# Autodesk Inventor assembly: Selection_Assy 2 Lanes
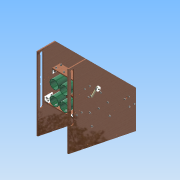
[picture p0: Inventor's stored thumbnail of the model, 180x180]
Saved by Autodesk Inventor 2018.1 (Build 221171000, 171)
## iProperties
Created: 2019-02-07
Part Number: Selection_Assy 2 Lanes
Document SubType Name: Assembly
Designer: James
Author: James
## Documents named in this file (24)
- C:\Users\admin\Desktop\Ball-Machine\Selection Sort\Selection - 2 Lanes\Selection_Assy 2 Lanes.iam
- C:\Users\admin\Desktop\Ball-Machine\Selection Sort\Selection_LHS.ipt
- C:\Users\admin\Desktop\Ball-Machine\Timing Gate\SAFL212 Oval 2 Bolt Flanged Unit.ipt
- C:\Users\admin\Desktop\Ball-Machine\Timing Gate\Nyloc Nut - M4.ipt
- C:\Users\admin\Desktop\Ball-Machine\Timing Gate\Socket Cap Screw - Standard - (A2) - M4 x 16.ipt
- C:\Users\admin\Desktop\Ball-Machine\Selection Sort\Locknut - M3.ipt
- C:\Users\admin\Desktop\Ball-Machine\Selection Sort\Socket Cap Screw - Standard - (A2) - M3 x 16.ipt
- C:\Users\admin\Desktop\Ball-Machine\Selection Sort\Selection_Lever 1.ipt
- C:\Users\admin\Desktop\Ball-Machine\Selection Sort\Socket Cap Screw - Standard - (A2) - M4 x 20.ipt
- C:\Users\admin\Desktop\Ball-Machine\Selection Sort\Selection_Lever Mount Piece.ipt
- C:\Users\admin\Desktop\Ball-Machine\Selection Sort\Socket Cap Screw - Standard - (A2) - M3 x 8.ipt
- C:\Users\admin\Desktop\Ball-Machine\Selection Sort\Selection_Washer.ipt
- C:\Users\admin\Desktop\Ball-Machine\Selection Sort\Selection_Gear 1.ipt
- C:\Users\admin\Desktop\Ball-Machine\Selection Sort\Selection_Lever 3.ipt
- C:\Users\admin\Desktop\Ball-Machine\Selection Sort\Selection_Counterweight.ipt
- C:\Users\admin\Desktop\Ball-Machine\Selection Sort\M3 x 20 - Hex. Head Set Screw (MS).ipt
- C:\Users\admin\Desktop\Ball-Machine\Selection Sort\Selection_Weight.ipt
- C:\Users\admin\Desktop\Ball-Machine\Selection Sort\Selection_Lever 2.ipt
- C:\Users\admin\Desktop\Ball-Machine\Selection Sort\Selection_Wire.ipt
- C:\Users\admin\Desktop\Ball-Machine\Selection Sort\Selection - 2 Lanes\Selection_Ramp 1 2 Lanes.iam
- C:\Users\admin\Desktop\Ball-Machine\Selection Sort\Selection - 2 Lanes\Selection_Exit Pipe Assy 2 Lanes.iam
- C:\Users\admin\Desktop\Ball-Machine\Selection Sort\Selection - 2 Lanes\Selection_Shaft Assy 2 Lanes.iam
- C:\Users\admin\Desktop\Ball-Machine\Timing Gate\Timing - 2 Lanes\Timing_Assy 2 Lanes.iam
- C:\Users\admin\Desktop\Ball-Machine\Selection Sort\Selection - 2 Lanes\Selection_Exit Pipe Assy Long 2 Lanes.iam
## Components (101 placed, 23 different names)
1. Selection_LHS:1 — Flush:1, Flush:2, Flush:3, Mate:4, Flush:9, Flush:10, Mate:37, Mate:38, Mate:39, Mate:42, Mate:43, Mate:56, Mate:70, Mate:71, Mate:116, Mate:117, Mate:118, Mate:119, Mate:120, Mate:121, Mate:128, Mate:129, Mate:131, Mate:152, Mate:155, Mate:193, Mate:194, Mate:195, Mate:196, Mate:200, Mate:203, Mate:204, Mate:205, Mate:206, Mate:207, Mate:208, Mate:210, Mate:211, Mate:213, Mate:214, Mate:225, Mate:226, Mate:227, Mate:228, Mate:232, Mate:233, Mate:234
2. Selection_Ramp 1 2 Lanes:1 [sub-assembly] — Flush:7, Mate:9, Mate:74, Mate:75, Mate:80, Mate:81, Mate:86, Mate:87, Mate:96, Mate:97, Mate:98, Mate:99
3. Selection_Ramp 1 2 Lanes:2 [sub-assembly] — Mate:4, Mate:76, Mate:77, Mate:82, Mate:83, Mate:88, Mate:89, Mate:94, Mate:95, Mate:102, Mate:103
4. Selection_Ramp 1 2 Lanes:3 [sub-assembly] — Flush:8, Mate:78, Mate:79, Mate:84, Mate:85, Mate:90, Mate:91, Mate:92, Mate:93, Mate:100, Mate:101
5. Selection_LHS:2 — Mate:9, Flush:9, Flush:10, Mate:52, Mate:53, Mate:54, Mate:55, Mate:57, Mate:62, Mate:63, Mate:74, Mate:75, Mate:76, Mate:77, Mate:78, Mate:79, Mate:104, Mate:105, Mate:106, Mate:107, Mate:108, Mate:109, Mate:132, Mate:134, Mate:135, Mate:148, Mate:149, Mate:159, Mate:160, Mate:161, Mate:162, Mate:163, Mate:164, Mate:189, Mate:190, Mate:191, Mate:192, Mate:197
6. Timing_Assy 2 Lanes:1 [sub-assembly] — Mate:36, Mate:37, Mate:38, Mate:39, Mate:40, Mate:41, Mate:44, Mate:45, Mate:48, Mate:49, Mate:50, Mate:51, Mate:56, Mate:57, Mate:58, Mate:59, Mate:60, Mate:61, Mate:66, Mate:67, Mate:68, Mate:69, Mate:219, Mate:220
7. SAFL212 Oval 2 Bolt Flanged Unit:3 — Mate:128, Mate:129, Mate:131, Mate:150, Mate:151, Mate:153, Mate:154, Mate:198
8. SAFL212 Oval 2 Bolt Flanged Unit:4 — Mate:132, Mate:134, Mate:135, Mate:144, Mate:145, Mate:146, Mate:147
9. Selection_Exit Pipe Assy Long 2 Lanes:1 [sub-assembly] — Mate:162, Mate:163, Mate:164, Mate:175, Mate:176, Mate:177, Mate:178, Mate:181, Mate:182, Mate:183, Mate:184
10. Selection_Exit Pipe Assy 2 Lanes:2 [sub-assembly] — Mate:159, Mate:160, Mate:161, Mate:173, Mate:174, Mate:179, Mate:180, Mate:185, Mate:186, Mate:187, Mate:188
11. Selection_Shaft Assy 2 Lanes:1 [sub-assembly] — Mate:197, Flush:11, Mate:198, Mate:247, Mate:248, Angle:1, Angle:2, Mate:249, Mate:250, Angle:3
12. Selection_Lever 1:1 — Mate:200, Mate:209, Mate:212, Flush:12, Mate:252, Flush:13
13. Selection_Lever Mount Piece:1 — Mate:209, Mate:210, Mate:211, Mate:212, Mate:215, Mate:216, Mate:217
14. Selection_Washer:1 — Mate:216, Mate:217, Mate:218
15. Selection_Gear 1:1 — Mate:219, Mate:220
16. Selection_Lever Mount Piece:2 — Mate:226, Mate:228, Mate:229, Mate:230
17. Socket Cap Screw - Standard - (A2) - M3 x 8:3 — Mate:225, Mate:227
18. Socket Cap Screw - Standard - (A2) - M3 x 8:4
19. Selection_Washer:2
20. Selection_Lever 3:1 — Mate:229, Mate:230, Tangent:3, Mate:251
21. Locknut - M3:9 — Mate:234
22. Socket Cap Screw - Standard - (A2) - M3 x 16:9 — Mate:232, Mate:233, Tangent:3
23. Selection_Counterweight:1 — Mate:235, Mate:236, Mate:242, Mate:247, Mate:248, Angle:1, Angle:2
24. Hex. Head Set Screw (MS) - M3 x 10:1 — Mate:235, Mate:236, Mate:237, Mate:238, Mate:239, Mate:240, Mate:241
25. Selection_Weight:1 — Mate:241, Mate:242, Mate:243
26. Selection_Weight:2 — Mate:240, Mate:243, Mate:244
27. Selection_Weight:3 — Mate:239, Mate:245, Mate:246
28. Selection_Weight:4 — Mate:238, Mate:244, Mate:245
29. Locknut - M3:10 — Mate:237, Mate:246
30. Selection_Lever 2:1 — Mate:249, Mate:250, Flush:12, Angle:3, Tangent:6, Tangent:7
31. Selection_Wire:1 — Mate:251, Mate:252, Flush:13
32. Socket Cap Screw - Standard - (A2) - M3 x 8:2 — Mate:215, Mate:218
33. Socket Cap Screw - Standard - (A2) - M3 x 8:1 — Mate:213, Mate:214
34. Nyloc Nut - M4:25 — Mate:207
35. Socket Cap Screw - Standard - (A2) - M4 x 20:2 — Mate:203, Mate:204, Tangent:6
36. Nyloc Nut - M4:26 — Mate:208
37. Socket Cap Screw - Standard - (A2) - M4 x 20:1 — Mate:205, Mate:206, Tangent:7
38. Nyloc Nut - M4:17 — Mate:173, Mate:179
39. Socket Cap Screw - Standard - (A2) - M4 x 16:17 — Mate:195
40. Nyloc Nut - M4:18 — Mate:174, Mate:180
41. Socket Cap Screw - Standard - (A2) - M4 x 16:18 — Mate:196
42. Nyloc Nut - M4:19 — Mate:175, Mate:176
43. Socket Cap Screw - Standard - (A2) - M4 x 16:19 — Mate:193
44. Nyloc Nut - M4:20 — Mate:177, Mate:178
45. Socket Cap Screw - Standard - (A2) - M4 x 16:20 — Mate:194
46. Nyloc Nut - M4:21 — Mate:181, Mate:183
47. Socket Cap Screw - Standard - (A2) - M4 x 16:21 — Mate:189
48. Nyloc Nut - M4:22 — Mate:182, Mate:184
49. Socket Cap Screw - Standard - (A2) - M4 x 16:22 — Mate:190
50. Nyloc Nut - M4:23 — Mate:185, Mate:188
51. Socket Cap Screw - Standard - (A2) - M4 x 16:23 — Mate:192
52. Nyloc Nut - M4:24 — Mate:186, Mate:187
53. Socket Cap Screw - Standard - (A2) - M4 x 16:24 — Mate:191
54. Locknut - M3:5 — Mate:149
55. Socket Cap Screw - Standard - (A2) - M3 x 16:5 — Mate:144, Mate:145
56. Locknut - M3:6 — Mate:148
57. Socket Cap Screw - Standard - (A2) - M3 x 16:6 — Mate:146, Mate:147
58. Locknut - M3:7 — Mate:152
59. Socket Cap Screw - Standard - (A2) - M3 x 16:7 — Mate:150, Mate:151
60. Locknut - M3:8 — Mate:155
61. Socket Cap Screw - Standard - (A2) - M3 x 16:8 — Mate:153, Mate:154
62. Nyloc Nut - M4:1 — Mate:44, Mate:46
63. Socket Cap Screw - Standard - (A2) - M4 x 16:1 — Mate:41, Mate:43, Mate:47
64. Nyloc Nut - M4:2 — Mate:45, Mate:47
65. Socket Cap Screw - Standard - (A2) - M4 x 16:2 — Mate:40, Mate:42, Mate:46
66. Nyloc Nut - M4:3 — Mate:49, Mate:50
67. Socket Cap Screw - Standard - (A2) - M4 x 16:3 — Mate:53, Mate:54
68. Nyloc Nut - M4:4 — Mate:48, Mate:51
69. Socket Cap Screw - Standard - (A2) - M4 x 16:4 — Mate:52, Mate:55
70. Locknut - M3:1 — Mate:62, Mate:64
71. Socket Cap Screw - Standard - (A2) - M3 x 16:1 — Mate:58, Mate:60, Mate:64
72. Locknut - M3:2 — Mate:63, Mate:65
73. Socket Cap Screw - Standard - (A2) - M3 x 16:2 — Mate:59, Mate:61, Mate:65
74. Locknut - M3:3 — Mate:70, Mate:72
75. Socket Cap Screw - Standard - (A2) - M3 x 16:3 — Mate:66, Mate:67, Mate:72
76. Locknut - M3:4 — Mate:71, Mate:73
77. Socket Cap Screw - Standard - (A2) - M3 x 16:4 — Mate:68, Mate:69, Mate:73
78. Nyloc Nut - M4:5 — Mate:104, Mate:110
79. Socket Cap Screw - Standard - (A2) - M4 x 16:5 — Mate:80, Mate:98, Mate:110
80. Nyloc Nut - M4:6 — Mate:105, Mate:112
81. Socket Cap Screw - Standard - (A2) - M4 x 16:6 — Mate:82, Mate:103, Mate:112
82. Nyloc Nut - M4:7 — Mate:106, Mate:115
83. Socket Cap Screw - Standard - (A2) - M4 x 16:7 — Mate:83, Mate:102, Mate:113
84. Nyloc Nut - M4:8 — Mate:107, Mate:113
85. Socket Cap Screw - Standard - (A2) - M4 x 16:8 — Mate:84, Mate:101, Mate:115
86. Nyloc Nut - M4:9 — Mate:108, Mate:111
87. Socket Cap Screw - Standard - (A2) - M4 x 16:9 — Mate:90, Mate:92, Mate:125
88. Nyloc Nut - M4:10 — Mate:109, Mate:114
89. Socket Cap Screw - Standard - (A2) - M4 x 16:10 — Mate:85, Mate:100, Mate:114
90. Nyloc Nut - M4:11 — Mate:116, Mate:124
91. Socket Cap Screw - Standard - (A2) - M4 x 16:11 — Mate:81, Mate:99, Mate:111
92. Nyloc Nut - M4:12 — Mate:117, Mate:126
93. Socket Cap Screw - Standard - (A2) - M4 x 16:12 — Mate:86, Mate:96, Mate:122
94. Nyloc Nut - M4:13 — Mate:118, Mate:127
95. Socket Cap Screw - Standard - (A2) - M4 x 16:13 — Mate:87, Mate:97, Mate:124
96. Nyloc Nut - M4:14 — Mate:119, Mate:125
97. Socket Cap Screw - Standard - (A2) - M4 x 16:14 — Mate:88, Mate:95, Mate:123
98. Nyloc Nut - M4:15 — Mate:120, Mate:123
99. Socket Cap Screw - Standard - (A2) - M4 x 16:15 — Mate:89, Mate:94, Mate:127
100. Nyloc Nut - M4:16 — Mate:121, Mate:122
101. Socket Cap Screw - Standard - (A2) - M4 x 16:16 — Mate:91, Mate:93, Mate:126
## Relationships (225: Mate 209, Flush 10, Tangent 3, Angle 3)
- Flush:1: Selection_LHS:1
- Flush:2: Selection_LHS:1
- Flush:3: Selection_LHS:1
- Flush:7: Selection_Ramp 1 2 Lanes:1
- Mate:4: Selection_LHS:1 ↔ Selection_Ramp 1 2 Lanes:2
- Flush:8: Selection_Ramp 1 2 Lanes:3
- Mate:9: Selection_Ramp 1 2 Lanes:1 ↔ Selection_LHS:2
- Flush:9: Selection_LHS:1 ↔ Selection_LHS:2
- Flush:10: Selection_LHS:1 ↔ Selection_LHS:2
- Mate:36: Timing_Assy 2 Lanes:1
- Mate:37: Selection_LHS:1 ↔ Timing_Assy 2 Lanes:1
- Mate:38: Selection_LHS:1 ↔ Timing_Assy 2 Lanes:1
- Mate:39: Selection_LHS:1 ↔ Timing_Assy 2 Lanes:1
- Mate:40: Timing_Assy 2 Lanes:1 ↔ Socket Cap Screw - Standard - (A2) - M4 x 16:2
- Mate:41: Timing_Assy 2 Lanes:1 ↔ Socket Cap Screw - Standard - (A2) - M4 x 16:1
- Mate:42: Selection_LHS:1 ↔ Socket Cap Screw - Standard - (A2) - M4 x 16:2
- Mate:43: Selection_LHS:1 ↔ Socket Cap Screw - Standard - (A2) - M4 x 16:1
- Mate:44: Timing_Assy 2 Lanes:1 ↔ Nyloc Nut - M4:1
- Mate:45: Timing_Assy 2 Lanes:1 ↔ Nyloc Nut - M4:2
- Mate:46: Nyloc Nut - M4:1 ↔ Socket Cap Screw - Standard - (A2) - M4 x 16:2
- Mate:47: Socket Cap Screw - Standard - (A2) - M4 x 16:1 ↔ Nyloc Nut - M4:2
- Mate:48: Timing_Assy 2 Lanes:1 ↔ Nyloc Nut - M4:4
- Mate:49: Timing_Assy 2 Lanes:1 ↔ Nyloc Nut - M4:3
- Mate:50: Timing_Assy 2 Lanes:1 ↔ Nyloc Nut - M4:3
- Mate:51: Timing_Assy 2 Lanes:1 ↔ Nyloc Nut - M4:4
- Mate:52: Selection_LHS:2 ↔ Socket Cap Screw - Standard - (A2) - M4 x 16:4
- Mate:53: Selection_LHS:2 ↔ Socket Cap Screw - Standard - (A2) - M4 x 16:3
- Mate:54: Selection_LHS:2 ↔ Socket Cap Screw - Standard - (A2) - M4 x 16:3
- Mate:55: Selection_LHS:2 ↔ Socket Cap Screw - Standard - (A2) - M4 x 16:4
- Mate:56: Selection_LHS:1 ↔ Timing_Assy 2 Lanes:1
- Mate:57: Selection_LHS:2 ↔ Timing_Assy 2 Lanes:1
- Mate:58: Timing_Assy 2 Lanes:1 ↔ Socket Cap Screw - Standard - (A2) - M3 x 16:1
- Mate:59: Timing_Assy 2 Lanes:1 ↔ Socket Cap Screw - Standard - (A2) - M3 x 16:2
- Mate:60: Timing_Assy 2 Lanes:1 ↔ Socket Cap Screw - Standard - (A2) - M3 x 16:1
- Mate:61: Timing_Assy 2 Lanes:1 ↔ Socket Cap Screw - Standard - (A2) - M3 x 16:2
- Mate:62: Selection_LHS:2 ↔ Locknut - M3:1
- Mate:63: Selection_LHS:2 ↔ Locknut - M3:2
- Mate:64: Locknut - M3:1 ↔ Socket Cap Screw - Standard - (A2) - M3 x 16:1
- Mate:65: Locknut - M3:2 ↔ Socket Cap Screw - Standard - (A2) - M3 x 16:2
- Mate:66: Timing_Assy 2 Lanes:1 ↔ Socket Cap Screw - Standard - (A2) - M3 x 16:3
- Mate:67: Timing_Assy 2 Lanes:1 ↔ Socket Cap Screw - Standard - (A2) - M3 x 16:3
- Mate:68: Timing_Assy 2 Lanes:1 ↔ Socket Cap Screw - Standard - (A2) - M3 x 16:4
- Mate:69: Timing_Assy 2 Lanes:1 ↔ Socket Cap Screw - Standard - (A2) - M3 x 16:4
- Mate:70: Selection_LHS:1 ↔ Locknut - M3:3
- Mate:71: Selection_LHS:1 ↔ Locknut - M3:4
- Mate:72: Locknut - M3:3 ↔ Socket Cap Screw - Standard - (A2) - M3 x 16:3
- Mate:73: Locknut - M3:4 ↔ Socket Cap Screw - Standard - (A2) - M3 x 16:4
- Mate:74: Selection_Ramp 1 2 Lanes:1 ↔ Selection_LHS:2
- Mate:75: Selection_Ramp 1 2 Lanes:1 ↔ Selection_LHS:2
- Mate:76: Selection_Ramp 1 2 Lanes:2 ↔ Selection_LHS:2
- Mate:77: Selection_Ramp 1 2 Lanes:2 ↔ Selection_LHS:2
- Mate:78: Selection_Ramp 1 2 Lanes:3 ↔ Selection_LHS:2
- Mate:79: Selection_Ramp 1 2 Lanes:3 ↔ Selection_LHS:2
- Mate:80: Selection_Ramp 1 2 Lanes:1 ↔ Socket Cap Screw - Standard - (A2) - M4 x 16:5
- Mate:81: Selection_Ramp 1 2 Lanes:1 ↔ Socket Cap Screw - Standard - (A2) - M4 x 16:11
- Mate:82: Selection_Ramp 1 2 Lanes:2 ↔ Socket Cap Screw - Standard - (A2) - M4 x 16:6
- Mate:83: Selection_Ramp 1 2 Lanes:2 ↔ Socket Cap Screw - Standard - (A2) - M4 x 16:7
- Mate:84: Selection_Ramp 1 2 Lanes:3 ↔ Socket Cap Screw - Standard - (A2) - M4 x 16:8
- Mate:85: Selection_Ramp 1 2 Lanes:3 ↔ Socket Cap Screw - Standard - (A2) - M4 x 16:10
- Mate:86: Selection_Ramp 1 2 Lanes:1 ↔ Socket Cap Screw - Standard - (A2) - M4 x 16:12
- Mate:87: Selection_Ramp 1 2 Lanes:1 ↔ Socket Cap Screw - Standard - (A2) - M4 x 16:13
- Mate:88: Selection_Ramp 1 2 Lanes:2 ↔ Socket Cap Screw - Standard - (A2) - M4 x 16:14
- Mate:89: Selection_Ramp 1 2 Lanes:2 ↔ Socket Cap Screw - Standard - (A2) - M4 x 16:15
- Mate:90: Selection_Ramp 1 2 Lanes:3 ↔ Socket Cap Screw - Standard - (A2) - M4 x 16:9
- Mate:91: Selection_Ramp 1 2 Lanes:3 ↔ Socket Cap Screw - Standard - (A2) - M4 x 16:16
- Mate:92: Selection_Ramp 1 2 Lanes:3 ↔ Socket Cap Screw - Standard - (A2) - M4 x 16:9
- Mate:93: Selection_Ramp 1 2 Lanes:3 ↔ Socket Cap Screw - Standard - (A2) - M4 x 16:16
- Mate:94: Selection_Ramp 1 2 Lanes:2 ↔ Socket Cap Screw - Standard - (A2) - M4 x 16:15
- Mate:95: Selection_Ramp 1 2 Lanes:2 ↔ Socket Cap Screw - Standard - (A2) - M4 x 16:14
- Mate:96: Selection_Ramp 1 2 Lanes:1 ↔ Socket Cap Screw - Standard - (A2) - M4 x 16:12
- Mate:97: Selection_Ramp 1 2 Lanes:1 ↔ Socket Cap Screw - Standard - (A2) - M4 x 16:13
- Mate:98: Selection_Ramp 1 2 Lanes:1 ↔ Socket Cap Screw - Standard - (A2) - M4 x 16:5
- Mate:99: Selection_Ramp 1 2 Lanes:1 ↔ Socket Cap Screw - Standard - (A2) - M4 x 16:11
- Mate:100: Selection_Ramp 1 2 Lanes:3 ↔ Socket Cap Screw - Standard - (A2) - M4 x 16:10
- Mate:101: Selection_Ramp 1 2 Lanes:3 ↔ Socket Cap Screw - Standard - (A2) - M4 x 16:8
- Mate:102: Selection_Ramp 1 2 Lanes:2 ↔ Socket Cap Screw - Standard - (A2) - M4 x 16:7
- Mate:103: Selection_Ramp 1 2 Lanes:2 ↔ Socket Cap Screw - Standard - (A2) - M4 x 16:6
- Mate:104: Selection_LHS:2 ↔ Nyloc Nut - M4:5
- Mate:105: Selection_LHS:2 ↔ Nyloc Nut - M4:6
- Mate:106: Selection_LHS:2 ↔ Nyloc Nut - M4:7
- Mate:107: Selection_LHS:2 ↔ Nyloc Nut - M4:8
- Mate:108: Selection_LHS:2 ↔ Nyloc Nut - M4:9
- Mate:109: Selection_LHS:2 ↔ Nyloc Nut - M4:10
- Mate:110: Nyloc Nut - M4:5 ↔ Socket Cap Screw - Standard - (A2) - M4 x 16:5
- Mate:111: Nyloc Nut - M4:9 ↔ Socket Cap Screw - Standard - (A2) - M4 x 16:11
- Mate:112: Nyloc Nut - M4:6 ↔ Socket Cap Screw - Standard - (A2) - M4 x 16:6
- Mate:113: Socket Cap Screw - Standard - (A2) - M4 x 16:7 ↔ Nyloc Nut - M4:8
- Mate:114: Nyloc Nut - M4:10 ↔ Socket Cap Screw - Standard - (A2) - M4 x 16:10
- Mate:115: Nyloc Nut - M4:7 ↔ Socket Cap Screw - Standard - (A2) - M4 x 16:8
- Mate:116: Selection_LHS:1 ↔ Nyloc Nut - M4:11
- Mate:117: Selection_LHS:1 ↔ Nyloc Nut - M4:12
- Mate:118: Selection_LHS:1 ↔ Nyloc Nut - M4:13
- Mate:119: Selection_LHS:1 ↔ Nyloc Nut - M4:14
- Mate:120: Selection_LHS:1 ↔ Nyloc Nut - M4:15
- Mate:121: Selection_LHS:1 ↔ Nyloc Nut - M4:16
- Mate:122: Socket Cap Screw - Standard - (A2) - M4 x 16:12 ↔ Nyloc Nut - M4:16
- Mate:123: Socket Cap Screw - Standard - (A2) - M4 x 16:14 ↔ Nyloc Nut - M4:15
- Mate:124: Nyloc Nut - M4:11 ↔ Socket Cap Screw - Standard - (A2) - M4 x 16:13
- Mate:125: Socket Cap Screw - Standard - (A2) - M4 x 16:9 ↔ Nyloc Nut - M4:14
- Mate:126: Nyloc Nut - M4:12 ↔ Socket Cap Screw - Standard - (A2) - M4 x 16:16
- Mate:127: Nyloc Nut - M4:13 ↔ Socket Cap Screw - Standard - (A2) - M4 x 16:15
- Mate:128: Selection_LHS:1 ↔ SAFL212 Oval 2 Bolt Flanged Unit:3
- Mate:129: Selection_LHS:1 ↔ SAFL212 Oval 2 Bolt Flanged Unit:3
- Mate:131: Selection_LHS:1 ↔ SAFL212 Oval 2 Bolt Flanged Unit:3
- Mate:132: Selection_LHS:2 ↔ SAFL212 Oval 2 Bolt Flanged Unit:4
- Mate:134: Selection_LHS:2 ↔ SAFL212 Oval 2 Bolt Flanged Unit:4
- Mate:135: Selection_LHS:2 ↔ SAFL212 Oval 2 Bolt Flanged Unit:4
- [Mate]: Locknut - M3:5 ↔ Socket Cap Screw - Standard - (A2) - M3 x 16:5
- [Mate]: Locknut - M3:6 ↔ Socket Cap Screw - Standard - (A2) - M3 x 16:6
- [Mate]: Locknut - M3:7 ↔ Socket Cap Screw - Standard - (A2) - M3 x 16:7
- [Mate]: Locknut - M3:8 ↔ Socket Cap Screw - Standard - (A2) - M3 x 16:8
- Mate:144: SAFL212 Oval 2 Bolt Flanged Unit:4 ↔ Socket Cap Screw - Standard - (A2) - M3 x 16:5
- Mate:145: SAFL212 Oval 2 Bolt Flanged Unit:4 ↔ Socket Cap Screw - Standard - (A2) - M3 x 16:5
- Mate:146: SAFL212 Oval 2 Bolt Flanged Unit:4 ↔ Socket Cap Screw - Standard - (A2) - M3 x 16:6
- Mate:147: SAFL212 Oval 2 Bolt Flanged Unit:4 ↔ Socket Cap Screw - Standard - (A2) - M3 x 16:6
- Mate:148: Selection_LHS:2 ↔ Locknut - M3:6
- Mate:149: Selection_LHS:2 ↔ Locknut - M3:5
- Mate:150: SAFL212 Oval 2 Bolt Flanged Unit:3 ↔ Socket Cap Screw - Standard - (A2) - M3 x 16:7
- Mate:151: SAFL212 Oval 2 Bolt Flanged Unit:3 ↔ Socket Cap Screw - Standard - (A2) - M3 x 16:7
- Mate:152: Selection_LHS:1 ↔ Locknut - M3:7
- Mate:153: SAFL212 Oval 2 Bolt Flanged Unit:3 ↔ Socket Cap Screw - Standard - (A2) - M3 x 16:8
- Mate:154: SAFL212 Oval 2 Bolt Flanged Unit:3 ↔ Socket Cap Screw - Standard - (A2) - M3 x 16:8
- Mate:155: Selection_LHS:1 ↔ Locknut - M3:8
- Mate:159: Selection_LHS:2 ↔ Selection_Exit Pipe Assy 2 Lanes:2
- Mate:160: Selection_LHS:2 ↔ Selection_Exit Pipe Assy 2 Lanes:2
- Mate:161: Selection_LHS:2 ↔ Selection_Exit Pipe Assy 2 Lanes:2
- Mate:162: Selection_LHS:2 ↔ Selection_Exit Pipe Assy Long 2 Lanes:1
- Mate:163: Selection_LHS:2 ↔ Selection_Exit Pipe Assy Long 2 Lanes:1
- Mate:164: Selection_LHS:2 ↔ Selection_Exit Pipe Assy Long 2 Lanes:1
- [Mate]: Nyloc Nut - M4:17 ↔ Socket Cap Screw - Standard - (A2) - M4 x 16:17
- [Mate]: Nyloc Nut - M4:18 ↔ Socket Cap Screw - Standard - (A2) - M4 x 16:18
- [Mate]: Nyloc Nut - M4:19 ↔ Socket Cap Screw - Standard - (A2) - M4 x 16:19
- [Mate]: Nyloc Nut - M4:20 ↔ Socket Cap Screw - Standard - (A2) - M4 x 16:20
- [Mate]: Nyloc Nut - M4:21 ↔ Socket Cap Screw - Standard - (A2) - M4 x 16:21
- [Mate]: Nyloc Nut - M4:22 ↔ Socket Cap Screw - Standard - (A2) - M4 x 16:22
- [Mate]: Nyloc Nut - M4:23 ↔ Socket Cap Screw - Standard - (A2) - M4 x 16:23
- [Mate]: Nyloc Nut - M4:24 ↔ Socket Cap Screw - Standard - (A2) - M4 x 16:24
- Mate:173: Selection_Exit Pipe Assy 2 Lanes:2 ↔ Nyloc Nut - M4:17
- Mate:174: Selection_Exit Pipe Assy 2 Lanes:2 ↔ Nyloc Nut - M4:18
- Mate:175: Selection_Exit Pipe Assy Long 2 Lanes:1 ↔ Nyloc Nut - M4:19
- Mate:176: Selection_Exit Pipe Assy Long 2 Lanes:1 ↔ Nyloc Nut - M4:19
- Mate:177: Selection_Exit Pipe Assy Long 2 Lanes:1 ↔ Nyloc Nut - M4:20
- Mate:178: Selection_Exit Pipe Assy Long 2 Lanes:1 ↔ Nyloc Nut - M4:20
- Mate:179: Selection_Exit Pipe Assy 2 Lanes:2 ↔ Nyloc Nut - M4:17
- Mate:180: Selection_Exit Pipe Assy 2 Lanes:2 ↔ Nyloc Nut - M4:18
- Mate:181: Selection_Exit Pipe Assy Long 2 Lanes:1 ↔ Nyloc Nut - M4:21
- Mate:182: Selection_Exit Pipe Assy Long 2 Lanes:1 ↔ Nyloc Nut - M4:22
- Mate:183: Selection_Exit Pipe Assy Long 2 Lanes:1 ↔ Nyloc Nut - M4:21
- Mate:184: Selection_Exit Pipe Assy Long 2 Lanes:1 ↔ Nyloc Nut - M4:22
- Mate:185: Selection_Exit Pipe Assy 2 Lanes:2 ↔ Nyloc Nut - M4:23
- Mate:186: Selection_Exit Pipe Assy 2 Lanes:2 ↔ Nyloc Nut - M4:24
- Mate:187: Selection_Exit Pipe Assy 2 Lanes:2 ↔ Nyloc Nut - M4:24
- Mate:188: Selection_Exit Pipe Assy 2 Lanes:2 ↔ Nyloc Nut - M4:23
- Mate:189: Selection_LHS:2 ↔ Socket Cap Screw - Standard - (A2) - M4 x 16:21
- Mate:190: Selection_LHS:2 ↔ Socket Cap Screw - Standard - (A2) - M4 x 16:22
- Mate:191: Selection_LHS:2 ↔ Socket Cap Screw - Standard - (A2) - M4 x 16:24
- Mate:192: Selection_LHS:2 ↔ Socket Cap Screw - Standard - (A2) - M4 x 16:23
- Mate:193: Selection_LHS:1 ↔ Socket Cap Screw - Standard - (A2) - M4 x 16:19
- Mate:194: Selection_LHS:1 ↔ Socket Cap Screw - Standard - (A2) - M4 x 16:20
- Mate:195: Selection_LHS:1 ↔ Socket Cap Screw - Standard - (A2) - M4 x 16:17
- Mate:196: Selection_LHS:1 ↔ Socket Cap Screw - Standard - (A2) - M4 x 16:18
- Mate:197: Selection_LHS:2 ↔ Selection_Shaft Assy 2 Lanes:1
- Flush:11: Selection_Shaft Assy 2 Lanes:1
- Mate:198: SAFL212 Oval 2 Bolt Flanged Unit:3 ↔ Selection_Shaft Assy 2 Lanes:1
- Mate:200: Selection_LHS:1 ↔ Selection_Lever 1:1
- [Mate]: Nyloc Nut - M4:25 ↔ Socket Cap Screw - Standard - (A2) - M4 x 20:2
- [Mate]: Nyloc Nut - M4:26 ↔ Socket Cap Screw - Standard - (A2) - M4 x 20:1
- Mate:203: Selection_LHS:1 ↔ Socket Cap Screw - Standard - (A2) - M4 x 20:2
- Mate:204: Selection_LHS:1 ↔ Socket Cap Screw - Standard - (A2) - M4 x 20:2
- Mate:205: Selection_LHS:1 ↔ Socket Cap Screw - Standard - (A2) - M4 x 20:1
- Mate:206: Selection_LHS:1 ↔ Socket Cap Screw - Standard - (A2) - M4 x 20:1
- Mate:207: Selection_LHS:1 ↔ Nyloc Nut - M4:25
- Mate:208: Selection_LHS:1 ↔ Nyloc Nut - M4:26
- Mate:209: Selection_Lever 1:1 ↔ Selection_Lever Mount Piece:1
- Mate:210: Selection_LHS:1 ↔ Selection_Lever Mount Piece:1
- Mate:211: Selection_LHS:1 ↔ Selection_Lever Mount Piece:1
- Mate:212 (0.5 mm): Selection_Lever 1:1 ↔ Selection_Lever Mount Piece:1
- Mate:213: Selection_LHS:1 ↔ Socket Cap Screw - Standard - (A2) - M3 x 8:1
- Mate:214: Selection_LHS:1 ↔ Socket Cap Screw - Standard - (A2) - M3 x 8:1
- Mate:215: Selection_Lever Mount Piece:1 ↔ Socket Cap Screw - Standard - (A2) - M3 x 8:2
- Mate:216: Selection_Lever Mount Piece:1 ↔ Selection_Washer:1
- Mate:217: Selection_Lever Mount Piece:1 ↔ Selection_Washer:1
- Mate:218: Selection_Washer:1 ↔ Socket Cap Screw - Standard - (A2) - M3 x 8:2
- Mate:219: Timing_Assy 2 Lanes:1 ↔ Selection_Gear 1:1
- Mate:220: Timing_Assy 2 Lanes:1 ↔ Selection_Gear 1:1
- [Mate]: Selection_Lever Mount Piece:2 ↔ Socket Cap Screw - Standard - (A2) - M3 x 8:4
- [Mate]: Selection_Lever Mount Piece:2 ↔ Selection_Washer:2
- [Mate]: Selection_Lever Mount Piece:2 ↔ Selection_Washer:2
- [Mate]: Socket Cap Screw - Standard - (A2) - M3 x 8:4 ↔ Selection_Washer:2
- Mate:225: Selection_LHS:1 ↔ Socket Cap Screw - Standard - (A2) - M3 x 8:3
- Mate:226: Selection_LHS:1 ↔ Selection_Lever Mount Piece:2
- Mate:227: Selection_LHS:1 ↔ Socket Cap Screw - Standard - (A2) - M3 x 8:3
- Mate:228: Selection_LHS:1 ↔ Selection_Lever Mount Piece:2
- Mate:229: Selection_Lever Mount Piece:2 ↔ Selection_Lever 3:1
- Mate:230: Selection_Lever Mount Piece:2 ↔ Selection_Lever 3:1
- [Mate]: Locknut - M3:9 ↔ Socket Cap Screw - Standard - (A2) - M3 x 16:9
- Mate:232: Selection_LHS:1 ↔ Socket Cap Screw - Standard - (A2) - M3 x 16:9
- Mate:233: Selection_LHS:1 ↔ Socket Cap Screw - Standard - (A2) - M3 x 16:9
- Mate:234: Selection_LHS:1 ↔ Locknut - M3:9
- Tangent:3: Selection_Lever 3:1 ↔ Socket Cap Screw - Standard - (A2) - M3 x 16:9
- Mate:235: Selection_Counterweight:1 ↔ Hex. Head Set Screw (MS) - M3 x 10:1
- Mate:236: Selection_Counterweight:1 ↔ Hex. Head Set Screw (MS) - M3 x 10:1
- Mate:237: Hex. Head Set Screw (MS) - M3 x 10:1 ↔ Locknut - M3:10
- Mate:238: Hex. Head Set Screw (MS) - M3 x 10:1 ↔ Selection_Weight:4
- Mate:239: Hex. Head Set Screw (MS) - M3 x 10:1 ↔ Selection_Weight:3
- Mate:240: Hex. Head Set Screw (MS) - M3 x 10:1 ↔ Selection_Weight:2
- Mate:241: Hex. Head Set Screw (MS) - M3 x 10:1 ↔ Selection_Weight:1
- Mate:242: Selection_Counterweight:1 ↔ Selection_Weight:1
- Mate:243: Selection_Weight:1 ↔ Selection_Weight:2
- Mate:244: Selection_Weight:2 ↔ Selection_Weight:4
- Mate:245: Selection_Weight:3 ↔ Selection_Weight:4
- Mate:246: Selection_Weight:3 ↔ Locknut - M3:10
- Mate:247: Selection_Shaft Assy 2 Lanes:1 ↔ Selection_Counterweight:1
- Mate:248: Selection_Shaft Assy 2 Lanes:1 ↔ Selection_Counterweight:1
- Angle:1 (-45 deg): Selection_Shaft Assy 2 Lanes:1 ↔ Selection_Counterweight:1
- Angle:2 (45 deg): Selection_Shaft Assy 2 Lanes:1 ↔ Selection_Counterweight:1
- Mate:249: Selection_Shaft Assy 2 Lanes:1 ↔ Selection_Lever 2:1
- Mate:250: Selection_Shaft Assy 2 Lanes:1 ↔ Selection_Lever 2:1
- Flush:12: Selection_Lever 1:1 ↔ Selection_Lever 2:1
- Angle:3 (0 deg): Selection_Shaft Assy 2 Lanes:1 ↔ Selection_Lever 2:1
- Tangent:6: Selection_Lever 2:1 ↔ Socket Cap Screw - Standard - (A2) - M4 x 20:2
- Tangent:7: Selection_Lever 2:1 ↔ Socket Cap Screw - Standard - (A2) - M4 x 20:1
- Mate:251: Selection_Lever 3:1 ↔ Selection_Wire:1
- Mate:252: Selection_Lever 1:1 ↔ Selection_Wire:1
- Flush:13 (-1 mm): Selection_Lever 1:1 ↔ Selection_Wire:1
## Named parameters: d159_d87 = 0 mm, d160_d87 = 0 mm, d161_d87 = 0 mm, d162_d87 = 0 mm, d190_d69 = 0 mm, d191_d69 = 0 mm, d192_d69 = 0 mm, d193_d69 = 0 mm, d194_d69 = 0 mm, d195_d69 = 0 mm, d196_d69 = 0 mm, d197_d69 = 0 mm, d227_d196_d69 = 0 mm, d228_d196_d69 = 0 mm, d254_d248 = 0 mm, d255_d249 = 0 mm, d256_d250 = 0 mm, d257_d251 = 0 mm, d264_d159_d87 = 0 mm
